# Autodesk Inventor assembly: ModuleAssembly
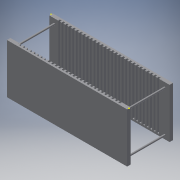
[picture p0: Inventor's stored thumbnail of the model, 180x180]
Saved by Autodesk Inventor 2016 (Build 200138000, 138)
## iProperties
Created: 2017-01-25
Part Number: ModuleAssembly
Document SubType Name: Assembly
Designer: RoboticsUser
Author: RoboticsUser
## Documents named in this file (3)
- C:\Robotics\CAD\2016-17_CAD\ModuleAssembly.iam
- C:\Robotics\CAD\2016-17_CAD\ModuleHolderReal.ipt
- C:\Robotics\CAD\2016-17_CAD\ModuleHolderBar.ipt
## Components (6 placed, 2 different names)
1. ModuleHolderReal:1 — Flush:1, Flush:2, Mate:1, Mate:2
2. ModuleHolderReal:2 — Flush:1, Flush:2, Mate:1, Tangent:1, Tangent:2
3. ModuleHolderBar:1 — Mate:2, Tangent:1, Tangent:2
4. ModuleHolderBar:5
5. ModuleHolderBar:6
6. ModuleHolderBar:7
## Component patterns: (2 elements), (2 elements, first: ModuleHolderBar:1), Component Pattern 1:2 (2 elements)
## Relationships (6: Flush 2, Mate 2, Tangent 2)
- Flush:1: ModuleHolderReal:1 ↔ ModuleHolderReal:2
- Flush:2: ModuleHolderReal:1 ↔ ModuleHolderReal:2
- Mate:1 (69.85 mm): ModuleHolderReal:1 ↔ ModuleHolderReal:2
- Mate:2: ModuleHolderReal:1 ↔ ModuleHolderBar:1
- Tangent:1 (-10.16 mm): ModuleHolderReal:2 ↔ ModuleHolderBar:1
- Tangent:2 (-10.16 mm): ModuleHolderReal:2 ↔ ModuleHolderBar:1
